# Autodesk Inventor assembly: Фильтр D1200
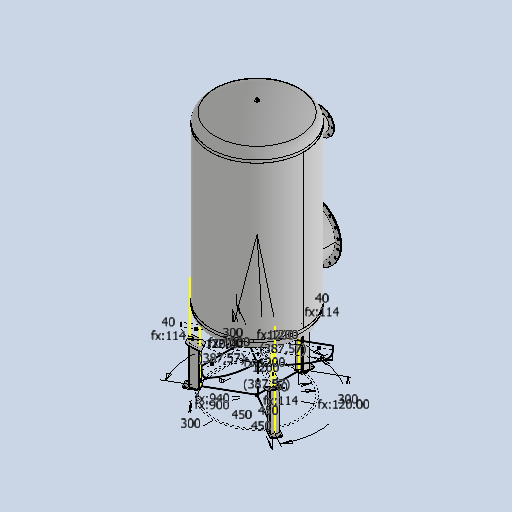
[picture p0: Inventor's stored thumbnail of the model, 512x512]
Saved by Autodesk Inventor 2025.1 (Build 291241020, 241B)
## iProperties
Created: 2025-02-13
Part Number: Фильтр D1200
Document SubType Name: Assembly
Designer: pokla
Author: pokla
Revision Number: 3
## Documents named in this file (15)
- C:\Users\user\YandexDisk-badmisterfox\home pc\Inventor\Pressure-filters\Filter D1000\ASY PNS- Filter column D1000.iam
- C:\Users\user\YandexDisk-badmisterfox\home pc\Inventor\Pressure-filters\D1200\PNS-621 charging hatch D1200.ipt
- C:\Users\user\YandexDisk-badmisterfox\home pc\Inventor\Pressure-filters\D1200\PNS-631 charging flange.ipt
- C:\Users\user\YandexDisk-badmisterfox\home pc\Inventor\Pressure-filters\D1200\PNS-612 accses hatch flangeipt.ipt
- C:\Users\user\YandexDisk-badmisterfox\home pc\Inventor\Pressure-filters\D1200\000 DIM PNS600-Filter column D1200.ipt
- C:\Users\user\YandexDisk-badmisterfox\home pc\Inventor\Pressure-filters\D1200\PNS-611 accses hatch tube.ipt
- C:\Users\user\YandexDisk-badmisterfox\home pc\Inventor\Pressure-filters\D1200\PNS-601 main tube D1000.ipt
- C:\Users\user\YandexDisk-badmisterfox\home pc\Inventor\Pressure-filters\D1200\PNS- 652 tube.ipt
- C:\Users\user\YandexDisk-badmisterfox\home pc\Inventor\Pressure-filters\D1200\PNS-633 charging blind flange.ipt
- C:\Users\user\YandexDisk-badmisterfox\home pc\Inventor\Pressure-filters\D1200\PNS - 604 dished head D1200.ipt
- C:\Users\user\YandexDisk-badmisterfox\home pc\Inventor\Pressure-filters\D1200\Fitting G1.ipt
- C:\Users\user\YandexDisk-badmisterfox\home pc\Inventor\Pressure-filters\D1200\PNS- 623 charging half tube.ipt
- C:\Users\user\YandexDisk-badmisterfox\home pc\Inventor\Pressure-filters\CC\en-US\DIN 2576 PN 10(2)\DIN 2576 Slip-On Flange for Welding Series 1 (ISO) - PN 10 500 x 508.ipt
- C:\Users\user\YandexDisk-badmisterfox\home pc\Inventor\Pressure-filters\D1200\ASY PNS680-Filter legs D1200.iam
- C:\Users\user\YandexDisk-badmisterfox\home pc\Inventor\Pressure-filters\CC\en-US\DIN 2576 PN 10(2)\DIN 2576 Slip-On Flange for Welding Series 1 (ISO) - PN 10 80 x 88.9.ipt
## Components (23 placed, 14 different names)
1. 000 DIM PNS600-Filter column D1200.ipt:1
2. PNS-621 charging hatch D1200.ipt:1 — Rigid:29
3. PNS-631 charging flange.ipt:1 — Rigid:22
4. PNS-612 accses hatch flangeipt.ipt:1 — Rigid:24, Rigid:25, Rigid:27, Rigid:28
5. PNS-611 accses hatch tube.ipt:1 — Rigid:10, Rigid:27
6. PNS-601 main tube D1000.ipt:1 — Rigid:10, Rigid:13, Rigid:14, Rigid:19, Rigid:20, Mate:1, Mate:2, Rigid:31, Rigid:30
7. PNS- 652 tube.ipt:1 — Rigid:31, Rotational:2
8. PNS-612 accses hatch flangeipt.ipt:2 — Rigid:24, Rigid:26
9. PNS-633 charging blind flange.ipt:1 — Rigid:21
10. PNS- 652 tube.ipt:2 — Rigid:30, Rotational:1
11. PNS - 604 dished head D1200.ipt:1 — Rigid:13, Rigid:16
12. PNS - 604 dished head D1200.ipt:2 — Rigid:14, Rigid:15, Mate:3
13. Fitting G1.ipt:1 — Rigid:15
14. Fitting G1.ipt:2 — Rigid:16
15. PNS- 623 charging half tube.ipt:1 — Rigid:19, Rigid:21, Rigid:22, Rigid:23
16. PNS- 623 charging half tube.ipt:2 — Rigid:20
17. PNS-633 charging blind flange.ipt:2 — Rigid:23
18. DIN 2576 Slip-On Flange for Welding Series 1 (ISO) - PN 10 500 x 508.ipt:1 — Rigid:28
19. PNS-612 accses hatch flangeipt.ipt:3 — Rigid:25, Rigid:29
20. PNS-612 accses hatch flangeipt.ipt:4 — Rigid:26
21. ASY PNS680-Filter legs D1200.iam:1 [sub-assembly] — Flush:1, Flush:2, Flush:3
22. DIN 2576 Slip-On Flange for Welding Series 1 (ISO) - PN 10 80 x 88.9.ipt:1 — Rotational:2
23. DIN 2576 Slip-On Flange for Welding Series 1 (ISO) - PN 10 80 x 88.9.ipt:2 — Rotational:1
## Relationships (26: WeldJoint 18, Mate 3, Flush 3, RevoluteJoint 2)
- Rigid:10 [WeldJoint] (66 mm): PNS-611 accses hatch tube.ipt:1 ↔ PNS-601 main tube D1000.ipt:1
- Rigid:13 [WeldJoint]: PNS-601 main tube D1000.ipt:1 ↔ PNS - 604 dished head D1200.ipt:1
- Rigid:14 [WeldJoint]: PNS-601 main tube D1000.ipt:1 ↔ PNS - 604 dished head D1200.ipt:2
- Rigid:15 [WeldJoint]: PNS - 604 dished head D1200.ipt:2 ↔ Fitting G1.ipt:1
- Rigid:16 [WeldJoint]: PNS - 604 dished head D1200.ipt:1 ↔ Fitting G1.ipt:2
- Rigid:19 [WeldJoint]: PNS-601 main tube D1000.ipt:1 ↔ PNS- 623 charging half tube.ipt:1
- Rigid:20 [WeldJoint]: PNS-601 main tube D1000.ipt:1 ↔ PNS- 623 charging half tube.ipt:2
- Rigid:21 [WeldJoint]: PNS-633 charging blind flange.ipt:1 ↔ PNS- 623 charging half tube.ipt:1
- Rigid:22 [WeldJoint]: PNS-631 charging flange.ipt:1 ↔ PNS- 623 charging half tube.ipt:1
- Rigid:23 [WeldJoint]: PNS- 623 charging half tube.ipt:1 ↔ PNS-633 charging blind flange.ipt:2
- Rigid:24 [WeldJoint]: PNS-612 accses hatch flangeipt.ipt:1 ↔ PNS-612 accses hatch flangeipt.ipt:2
- Rigid:25 [WeldJoint]: PNS-612 accses hatch flangeipt.ipt:1 ↔ PNS-612 accses hatch flangeipt.ipt:3
- Rigid:26 [WeldJoint]: PNS-612 accses hatch flangeipt.ipt:2 ↔ PNS-612 accses hatch flangeipt.ipt:4
- Rigid:27 [WeldJoint]: PNS-612 accses hatch flangeipt.ipt:1 ↔ PNS-611 accses hatch tube.ipt:1
- Rigid:28 [WeldJoint]: PNS-612 accses hatch flangeipt.ipt:1 ↔ DIN 2576 Slip-On Flange for Welding Series 1 (ISO) - PN 10 500 x 508.ipt:1
- Mate:1: PNS-601 main tube D1000.ipt:1
- Mate:2: PNS-601 main tube D1000.ipt:1
- Mate:3 (2750 mm): PNS - 604 dished head D1200.ipt:2
- Flush:1: ASY PNS680-Filter legs D1200.iam:1
- Flush:2: ASY PNS680-Filter legs D1200.iam:1
- Flush:3: ASY PNS680-Filter legs D1200.iam:1
- Rigid:29 [WeldJoint]: PNS-621 charging hatch D1200.ipt:1 ↔ PNS-612 accses hatch flangeipt.ipt:3
- Rigid:31 [WeldJoint]: PNS-601 main tube D1000.ipt:1 ↔ PNS- 652 tube.ipt:1
- Rigid:30 [WeldJoint]: PNS-601 main tube D1000.ipt:1 ↔ PNS- 652 tube.ipt:2
- Rotational:1 [RevoluteJoint]: PNS- 652 tube.ipt:2 ↔ DIN 2576 Slip-On Flange for Welding Series 1 (ISO) - PN 10 80 x 88.9.ipt:2
- Rotational:2 [RevoluteJoint]: PNS- 652 tube.ipt:1 ↔ DIN 2576 Slip-On Flange for Welding Series 1 (ISO) - PN 10 80 x 88.9.ipt:1
